# Autodesk Inventor assembly: ASY TZS 1480 Filter legs
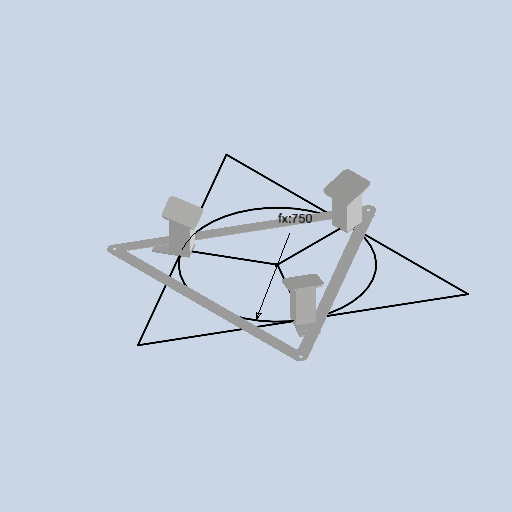
[picture p0: Inventor's stored thumbnail of the model, 512x512]
Saved by Autodesk Inventor 2025 (Build 290162010, 162A)
## iProperties
Created: 2025-02-20
Part Number: ASY TZS 1480 Filter legs
Document SubType Name: Assembly
Designer: user
Author: user
## Documents named in this file (6)
- C:\Users\pokla\Documents\Inventor\TZS-Tazovskiy\ASY TZS 1480 Filter legs.iam
- C:\Users\pokla\Documents\Inventor\TZS-Tazovskiy\TZS 1481 leg sketch.ipt
- C:\Users\pokla\Documents\Inventor\TZS-Tazovskiy\TZS 1782 leg plate for filter.ipt
- C:\Users\pokla\Documents\Inventor\TZS-Tazovskiy\TZS 1483 leg floor plate.ipt
- C:\Users\pokla\Documents\Inventor\TZS-Tazovskiy\TZS 1489 leg D1200 pattern.ipt
- C:\Users\pokla\Documents\Inventor\TZS-Tazovskiy\TZS 1484 leg tube.ipt
## Components (11 placed, 5 different names)
1. TZS 1481 leg sketch.ipt:1 — Mate:1, Mate:2, Mate:3, Mate:4, Mate:5, Mate:6, Mate:7
2. TZS 1782 leg plate for filter.ipt:1 — Rigid:5
3. TZS 1782 leg plate for filter.ipt:2 — Rigid:4
4. TZS 1782 leg plate for filter.ipt:3 — Rigid:6
5. TZS 1483 leg floor plate.ipt:1 — Mate:1, Mate:2, Mate:3, Rigid:2
6. TZS 1483 leg floor plate.ipt:2 — Mate:4, Mate:5, Flush:1, Rigid:3
7. TZS 1483 leg floor plate.ipt:3 — Flush:2, Mate:6, Mate:7, Rigid:1
8. TZS 1489 leg D1200 pattern.ipt:1
9. TZS 1484 leg tube.ipt:1 — Rigid:1, Rigid:6
10. TZS 1484 leg tube.ipt:2 — Rigid:2, Rigid:5
11. TZS 1484 leg tube.ipt:3 — Rigid:3, Rigid:4
## Relationships (15: Mate 7, WeldJoint 6, Flush 2)
- Mate:1: TZS 1481 leg sketch.ipt:1 ↔ TZS 1483 leg floor plate.ipt:1
- Mate:2: TZS 1481 leg sketch.ipt:1 ↔ TZS 1483 leg floor plate.ipt:1
- Mate:3: TZS 1481 leg sketch.ipt:1 ↔ TZS 1483 leg floor plate.ipt:1
- Mate:4: TZS 1481 leg sketch.ipt:1 ↔ TZS 1483 leg floor plate.ipt:2
- Mate:5: TZS 1481 leg sketch.ipt:1 ↔ TZS 1483 leg floor plate.ipt:2
- Flush:1: TZS 1483 leg floor plate.ipt:2
- Flush:2: TZS 1483 leg floor plate.ipt:3
- Mate:6: TZS 1481 leg sketch.ipt:1 ↔ TZS 1483 leg floor plate.ipt:3
- Mate:7: TZS 1481 leg sketch.ipt:1 ↔ TZS 1483 leg floor plate.ipt:3
- Rigid:1 [WeldJoint]: TZS 1483 leg floor plate.ipt:3 ↔ TZS 1484 leg tube.ipt:1
- Rigid:2 [WeldJoint]: TZS 1483 leg floor plate.ipt:1 ↔ TZS 1484 leg tube.ipt:2
- Rigid:3 [WeldJoint]: TZS 1483 leg floor plate.ipt:2 ↔ TZS 1484 leg tube.ipt:3
- Rigid:4 [WeldJoint]: TZS 1782 leg plate for filter.ipt:2 ↔ TZS 1484 leg tube.ipt:3
- Rigid:5 [WeldJoint]: TZS 1782 leg plate for filter.ipt:1 ↔ TZS 1484 leg tube.ipt:2
- Rigid:6 [WeldJoint]: TZS 1782 leg plate for filter.ipt:3 ↔ TZS 1484 leg tube.ipt:1
